# Autodesk Inventor assembly: Leg
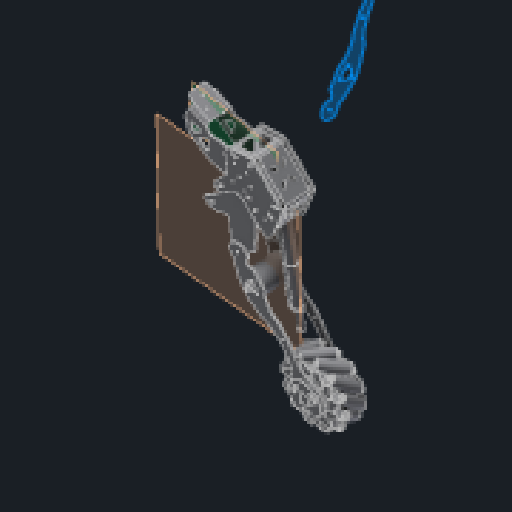
[picture p0: Inventor's stored thumbnail of the model, 512x512]
Saved by Autodesk Inventor 2025.2 (Build 292293000, 293)
## iProperties
Created: 2020-05-17
Part Number: Leg
Document SubType Name: Assembly
Designer: valer
Author: valer
## Documents named in this file (14)
- C:\Users\valer\Desktop\str1ker\cad\Leg.iam
- C:\Users\valer\Desktop\str1ker\cad\Knee.ipt
- C:\Users\valer\Desktop\str1ker\cad\LowerLeg.ipt
- C:\Users\valer\Desktop\str1ker\cad\UpperLeg.ipt
- C:\Users\valer\Desktop\str1ker\cad\Hip.ipt
- C:\Users\valer\Desktop\str1ker\cad\HipCoverTop.ipt
- C:\Users\valer\Desktop\str1ker\cad\external\FA-RMS-15-12-4-Piston.ipt
- C:\Users\valer\Desktop\str1ker\cad\external\FA-RMS-15-12-4.ipt
- C:\Users\valer\Desktop\str1ker\cad\external\2796N15_Omni-Directional Wheel.ipt
- C:\Users\valer\Desktop\str1ker\cad\external\MY6812-12VDC-120W-Motor.ipt
- C:\Users\valer\Desktop\str1ker\cad\external\SprocketMDEOOSKY-25H-47T.ipt
- C:\Users\valer\Desktop\str1ker\cad\LegHub.ipt
- C:\Users\valer\Desktop\str1ker\cad\external\6656K234_Ultra-Thin Ball Bearing.ipt
- C:\Users\valer\Desktop\str1ker\cad\LegInsideConnector.ipt
## Components (19 placed, 13 different names)
1. Knee:1 — Flush:1, Mate:1, Mate:4, Mate:68, Mate:112
2. UpperLeg:1 — Flush:1, Mate:1, Mate:4, Mate:6, Mate:7, Mate:17, Mate:18, Symmetry:1, Mate:61
3. Hip:1 — Mate:6, Mate:7, Mate:12, Mate:13, Mate:39
4. Knee:2 — Mate:79, Mate:115
5. UpperLeg:2 — Mate:12, Mate:13, Symmetry:1, Mate:36, Mate:60
6. HipCoverTop:1 — Mate:17, Mate:18, Mate:39, Mate:60, Mate:61, Mate:113, Mate:114, Mate:116, Mate:117
7. FA-RMS-15-12-4-Piston:1 — Mate:35, Mate:83
8. FA-RMS-15-12-4:1 — Mate:35, Mate:36
9. MY6812-12VDC-120W-Motor:1 — Mate:77, Mate:80, Mate:89, Mate:93, Flush:4, Flush:5
10. LowerLeg:3 — Mate:68, Mate:77, Mate:80, Mate:83, Mate:94
11. LowerLeg:4 — Mate:79, Mate:89, Mate:98, Mate:111
12. SprocketMDEOOSKY-25H-47T:1 — Flush:4, Mate:96, Mate:110, Flush:5
13. LegHub:1 — Mate:94, Mate:97, Mate:108, Mate:109, Mate:110
14. 2796N15_Omni-Directional Wheel:1 — Mate:96, Mate:97, Mate:98, Mate:102, Mate:103, Mate:104, Mate:105, Mate:106, Mate:107, Mate:108, Mate:109
15. 6656K234_Ultra-Thin Ball Bearing:1 — Mate:102, Mate:111
16. 6656K234_Ultra-Thin Ball Bearing:2 — Mate:103, Mate:104
17. LegHub:3 — Mate:105, Mate:106, Mate:107
18. LegInsideConnector:1 — Mate:112, Mate:113, Mate:114
19. LegInsideConnector:2 — Mate:115, Mate:116, Mate:117
## Relationships (47: Mate 42, Flush 4, Symmetry 1)
- Flush:1 (-5.08 mm): Knee:1 ↔ UpperLeg:1
- Mate:1: Knee:1 ↔ UpperLeg:1
- Mate:4: Knee:1 ↔ UpperLeg:1
- Mate:6: UpperLeg:1 ↔ Hip:1
- Mate:7: UpperLeg:1 ↔ Hip:1
- [Flush] (5.08 mm): Knee:2 ↔ UpperLeg:2
- [Mate]: Knee:2 ↔ UpperLeg:2
- [Mate]: Knee:2 ↔ UpperLeg:2
- Mate:12: Hip:1 ↔ UpperLeg:2
- Mate:13: Hip:1 ↔ UpperLeg:2
- Mate:17: UpperLeg:1 ↔ HipCoverTop:1
- Mate:18: UpperLeg:1 ↔ HipCoverTop:1
- Symmetry:1: UpperLeg:1 ↔ UpperLeg:2
- Mate:35: FA-RMS-15-12-4-Piston:1 ↔ FA-RMS-15-12-4:1
- Mate:36: UpperLeg:2 ↔ FA-RMS-15-12-4:1
- Mate:39: Hip:1 ↔ HipCoverTop:1
- Mate:60: UpperLeg:2 ↔ HipCoverTop:1
- Mate:61: UpperLeg:1 ↔ HipCoverTop:1
- Mate:68: Knee:1 ↔ LowerLeg:3
- Mate:77: MY6812-12VDC-120W-Motor:1 ↔ LowerLeg:3
- Mate:79: Knee:2 ↔ LowerLeg:4
- Mate:80: MY6812-12VDC-120W-Motor:1 ↔ LowerLeg:3
- Mate:83: FA-RMS-15-12-4-Piston:1 ↔ LowerLeg:3
- Mate:89: MY6812-12VDC-120W-Motor:1 ↔ LowerLeg:4
- Mate:93: MY6812-12VDC-120W-Motor:1
- Mate:94: LowerLeg:3 ↔ LegHub:1
- Flush:4: MY6812-12VDC-120W-Motor:1 ↔ SprocketMDEOOSKY-25H-47T:1
- Mate:96: SprocketMDEOOSKY-25H-47T:1 ↔ 2796N15_Omni-Directional Wheel:1
- Mate:97: LegHub:1 ↔ 2796N15_Omni-Directional Wheel:1
- Mate:98: LowerLeg:4 ↔ 2796N15_Omni-Directional Wheel:1
- Mate:102: 2796N15_Omni-Directional Wheel:1 ↔ 6656K234_Ultra-Thin Ball Bearing:1
- Mate:103: 2796N15_Omni-Directional Wheel:1 ↔ 6656K234_Ultra-Thin Ball Bearing:2
- Mate:104: 2796N15_Omni-Directional Wheel:1 ↔ 6656K234_Ultra-Thin Ball Bearing:2
- Mate:105: 2796N15_Omni-Directional Wheel:1 ↔ LegHub:3
- Mate:106: 2796N15_Omni-Directional Wheel:1 ↔ LegHub:3
- Mate:107: 2796N15_Omni-Directional Wheel:1 ↔ LegHub:3
- Mate:108: LegHub:1 ↔ 2796N15_Omni-Directional Wheel:1
- Mate:109: LegHub:1 ↔ 2796N15_Omni-Directional Wheel:1
- Mate:110: SprocketMDEOOSKY-25H-47T:1 ↔ LegHub:1
- Flush:5: MY6812-12VDC-120W-Motor:1 ↔ SprocketMDEOOSKY-25H-47T:1
- Mate:111: LowerLeg:4 ↔ 6656K234_Ultra-Thin Ball Bearing:1
- Mate:112: Knee:1 ↔ LegInsideConnector:1
- Mate:113: HipCoverTop:1 ↔ LegInsideConnector:1
- Mate:114: HipCoverTop:1 ↔ LegInsideConnector:1
- Mate:115: Knee:2 ↔ LegInsideConnector:2
- Mate:116: HipCoverTop:1 ↔ LegInsideConnector:2
- Mate:117: HipCoverTop:1 ↔ LegInsideConnector:2
## Named parameters: d11_d0 = 5.08 mm, d12_d1 = 0 mm, d15_d5 = 0 mm
